# Autodesk Inventor assembly: Subensamble_Base cortadora
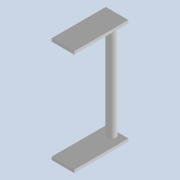
[picture p0: Inventor's stored thumbnail of the model, 180x180]
Saved by Autodesk Inventor 2021 (Build 250183000, 183)
## iProperties
Created: 2021-04-30
Part Number: Subensamble_Base cortadora
Document SubType Name: Assembly
Designer: Admin
Author: Admin
## Documents named in this file (3)
- C:\Users\Admin\OneDrive - Universidad Nacional de Colombia\Doceabo semestre\AUTO\proyecto Auto\Proyecto_APM\CADs estaciones a automatizar\Estación corte\Subensamble_Base cortadora.iam
- C:\Users\Admin\OneDrive - Universidad Nacional de Colombia\Doceabo semestre\AUTO\proyecto Auto\Proyecto_APM\CADs estaciones a automatizar\Estación corte\Base_cortadora.ipt
- C:\Users\Admin\OneDrive - Universidad Nacional de Colombia\Doceabo semestre\AUTO\proyecto Auto\Proyecto_APM\CADs estaciones a automatizar\Estación corte\Barra base cotadora.ipt
## Components (3 placed, 2 different names)
1. Base_cortadora:1 — Nivelación:1, De rotación:1
2. Base_cortadora:2 — Coincidencia:1, Nivelación:2
3. Barra base cotadora:1 — Nivelación:1, De rotación:1, Coincidencia:1, Nivelación:2
## Relationships (4: Flush 2, RevoluteJoint 1, Mate 1)
- Nivelación:1 [Flush]: Base_cortadora:1 ↔ Barra base cotadora:1
- De rotación:1 [RevoluteJoint]: Base_cortadora:1 ↔ Barra base cotadora:1
- Coincidencia:1 [Mate]: Base_cortadora:2 ↔ Barra base cotadora:1
- Nivelación:2 [Flush]: Base_cortadora:2 ↔ Barra base cotadora:1
